# Autodesk Inventor assembly: Boiler SubAssy
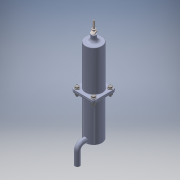
[picture p0: Inventor's stored thumbnail of the model, 180x180]
Saved by Autodesk Inventor 2018 (Build 220112000, 112)
## iProperties
Created: 2020-03-31
Part Number: Boiler SubAssy
Description: STEP AP214
Document SubType Name: Assembly
Designer: emile
Sending System: SolidWorks 2017
Preprocessor: SwSTEP 2.0
Title: Boiler SubAssy.STEP
Revision Number: ANY
## Documents named in this file (8)
- C:\Users\emile\OneDrive\Documents\GitHub\VentilatorCovid19\Respirator\MultiLine\boiler\Boiler SubAssy.iam
- C:\Users\emile\OneDrive\Documents\GitHub\VentilatorCovid19\Respirator\MultiLine\boiler\Boiler Bottom.ipt
- C:\Users\emile\OneDrive\Documents\GitHub\VentilatorCovid19\Respirator\MultiLine\boiler\Boiler Top.ipt
- C:\Users\emile\OneDrive\Documents\GitHub\VentilatorCovid19\Respirator\MultiLine\boiler\Seal.ipt
- C:\Users\emile\OneDrive\Documents\GitHub\VentilatorCovid19\Respirator\MultiLine\boiler\hex flange nut_am_B18.2.2.4M - Hex flange nut, M8 x 1.25 --N.ipt
- C:\Users\emile\OneDrive\Documents\GitHub\VentilatorCovid19\Respirator\MultiLine\boiler\flat washer narrow_am_B18.22M - Plain washer, 8 mm, narrow.ipt
- C:\Users\emile\OneDrive\Documents\GitHub\VentilatorCovid19\Respirator\MultiLine\boiler\formed hex screw_am_B18.2.3.2M - Formed hex screw, M8 x 1.25 x 30 --30WN.ipt
- C:\Users\emile\OneDrive\Documents\GitHub\VentilatorCovid19\Respirator\MultiLine\MedicalAirFilter\Vanamatic-4130.ipt
## Components (20 placed, 20 different names)
1. Boiler Bottom_1
2. Boiler Top_2 — Mate:3, Mate:4
3. Seal_3
4. hex flange nut_am_B18.2.2.4M - Hex flange nut, M8 x 1.25 --N_4
5. hex flange nut_am_B18.2.2.4M - Hex flange nut, M8 x 1.25 --N_5
6. hex flange nut_am_B18.2.2.4M - Hex flange nut, M8 x 1.25 --N_6
7. hex flange nut_am_B18.2.2.4M - Hex flange nut, M8 x 1.25 --N_7
8. flat washer narrow_am_B18.22M - Plain washer, 8 mm, narrow_8
9. flat washer narrow_am_B18.22M - Plain washer, 8 mm, narrow_9
10. flat washer narrow_am_B18.22M - Plain washer, 8 mm, narrow_10
11. flat washer narrow_am_B18.22M - Plain washer, 8 mm, narrow_11
12. flat washer narrow_am_B18.22M - Plain washer, 8 mm, narrow_12
13. flat washer narrow_am_B18.22M - Plain washer, 8 mm, narrow_13
14. flat washer narrow_am_B18.22M - Plain washer, 8 mm, narrow_14
15. flat washer narrow_am_B18.22M - Plain washer, 8 mm, narrow_15
16. formed hex screw_am_B18.2.3.2M - Formed hex screw, M8 x 1.25 x 30 --30WN_16
17. formed hex screw_am_B18.2.3.2M - Formed hex screw, M8 x 1.25 x 30 --30WN_17
18. formed hex screw_am_B18.2.3.2M - Formed hex screw, M8 x 1.25 x 30 --30WN_18
19. formed hex screw_am_B18.2.3.2M - Formed hex screw, M8 x 1.25 x 30 --30WN_19
20. Vanamatic-4130:1 — Mate:3, Mate:4
## Relationships (2: Mate 2)
- Mate:3: Boiler Top_2 ↔ Vanamatic-4130:1
- Mate:4 (3.175 mm): Boiler Top_2 ↔ Vanamatic-4130:1
